# Autodesk Inventor assembly: Bearing Block Assem
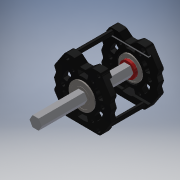
[picture p0: Inventor's stored thumbnail of the model, 180x180]
Saved by Autodesk Inventor 2018 (Build 220112000, 112)
## iProperties
Created: 2018-11-11
Part Number: Bearing Block Assem
Document SubType Name: Assembly
Designer: maste
Author: maste
## Documents named in this file (8)
- F:\Summer Drive Base V1\Summer Drivebase\Bearing Block Assem.iam
- F:\Summer Drive Base V1\Summer Drivebase\VersaBlock_Kit_217-3432.ipt
- F:\Summer Drive Base V1\Summer Drivebase\Ignore this-For constraining purposes.ipt
- F:\Summer Drive Base V1\Summer Drivebase\Pretend this is a bolt.ipt
- F:\Summer Drive Base V1\Summer Drivebase\0_500_Hex_ID_x_1_125_OD_x_0_313_WD_Flanged_Bearing_v2_217-3875.ipt
- F:\Summer Drive Base V1\Summer Drivebase\am-1238+Collar+Clamp,+0.5''+Hex+Bore,+Aluminum.iam
- F:\Summer Drive Base V1\Summer Drivebase\5-1875 hex shaft.ipt
- F:\Summer Drive Base V1\Summer Drivebase\0.125in Spacer.ipt
## Components (12 placed, 7 different names)
1. VersaBlock_Kit_217-3432:1 — Mate:4, Mate:5, Mate:6, Mate:7, Mate:8, Mate:11, Mate:13, Mate:15, Mate:16, Rotation:2
2. VersaBlock_Kit_217-3432:2 — Mate:1, Mate:2, Mate:3, Mate:9, Mate:10, Mate:12, Mate:14, Mate:19, Mate:20, Rotation:1
3. Ignore this-For constraining purposes:3 — Mate:1, Mate:2, Mate:3
4. Pretend this is a bolt:1 — Mate:7, Mate:8, Mate:9, Mate:10
5. Pretend this is a bolt:2 — Mate:11, Mate:12, Mate:13, Mate:14
6. Ignore this-For constraining purposes:4 — Mate:4, Mate:5, Mate:6
7. 0_500_Hex_ID_x_1_125_OD_x_0_313_WD_Flanged_Bearing_v2_217-3875:1 — Mate:15, Mate:16, Mate:17, Flush:1, Flush:2, Rotation:2
8. 0_500_Hex_ID_x_1_125_OD_x_0_313_WD_Flanged_Bearing_v2_217-3875:2 — Mate:18, Flush:3, Flush:4, Mate:19, Mate:20, Rotation:1, Mate:21, Flush:5, Flush:6
9. am-1238+Collar+Clamp,+0.5''+Hex+Bore,+Aluminum:1 [sub-assembly] — Mate:21, Flush:5, Flush:6, Flush:7, Mate:22, Mate:23
10. 5-1875 hex shaft:1 — Flush:7, Mate:22, Mate:23
11. 0.125in Spacer:1 — Mate:17, Flush:1, Flush:2
12. 0.125in Spacer:2 — Mate:18, Flush:3, Flush:4
## Relationships (32: Mate 23, Flush 7, RelateRotation 2)
- Mate:1: VersaBlock_Kit_217-3432:2 ↔ Ignore this-For constraining purposes:3
- Mate:2: VersaBlock_Kit_217-3432:2 ↔ Ignore this-For constraining purposes:3
- Mate:3: VersaBlock_Kit_217-3432:2 ↔ Ignore this-For constraining purposes:3
- Mate:4: VersaBlock_Kit_217-3432:1 ↔ Ignore this-For constraining purposes:4
- Mate:5: VersaBlock_Kit_217-3432:1 ↔ Ignore this-For constraining purposes:4
- Mate:6: VersaBlock_Kit_217-3432:1 ↔ Ignore this-For constraining purposes:4
- Mate:7: VersaBlock_Kit_217-3432:1 ↔ Pretend this is a bolt:1
- Mate:8: VersaBlock_Kit_217-3432:1 ↔ Pretend this is a bolt:1
- Mate:9: VersaBlock_Kit_217-3432:2 ↔ Pretend this is a bolt:1
- Mate:10: VersaBlock_Kit_217-3432:2 ↔ Pretend this is a bolt:1
- Mate:11: VersaBlock_Kit_217-3432:1 ↔ Pretend this is a bolt:2
- Mate:12: VersaBlock_Kit_217-3432:2 ↔ Pretend this is a bolt:2
- Mate:13: VersaBlock_Kit_217-3432:1 ↔ Pretend this is a bolt:2
- Mate:14: VersaBlock_Kit_217-3432:2 ↔ Pretend this is a bolt:2
- Mate:15: VersaBlock_Kit_217-3432:1 ↔ 0_500_Hex_ID_x_1_125_OD_x_0_313_WD_Flanged_Bearing_v2_217-3875:1
- Mate:16: VersaBlock_Kit_217-3432:1 ↔ 0_500_Hex_ID_x_1_125_OD_x_0_313_WD_Flanged_Bearing_v2_217-3875:1
- Mate:17: 0_500_Hex_ID_x_1_125_OD_x_0_313_WD_Flanged_Bearing_v2_217-3875:1 ↔ 0.125in Spacer:1
- Flush:1: 0_500_Hex_ID_x_1_125_OD_x_0_313_WD_Flanged_Bearing_v2_217-3875:1 ↔ 0.125in Spacer:1
- Flush:2: 0_500_Hex_ID_x_1_125_OD_x_0_313_WD_Flanged_Bearing_v2_217-3875:1 ↔ 0.125in Spacer:1
- Mate:18: 0_500_Hex_ID_x_1_125_OD_x_0_313_WD_Flanged_Bearing_v2_217-3875:2 ↔ 0.125in Spacer:2
- Flush:3: 0_500_Hex_ID_x_1_125_OD_x_0_313_WD_Flanged_Bearing_v2_217-3875:2 ↔ 0.125in Spacer:2
- Flush:4: 0_500_Hex_ID_x_1_125_OD_x_0_313_WD_Flanged_Bearing_v2_217-3875:2 ↔ 0.125in Spacer:2
- Mate:19: VersaBlock_Kit_217-3432:2 ↔ 0_500_Hex_ID_x_1_125_OD_x_0_313_WD_Flanged_Bearing_v2_217-3875:2
- Mate:20: VersaBlock_Kit_217-3432:2 ↔ 0_500_Hex_ID_x_1_125_OD_x_0_313_WD_Flanged_Bearing_v2_217-3875:2
- Rotation:1 [RelateRotation] (1 ul): VersaBlock_Kit_217-3432:2 ↔ 0_500_Hex_ID_x_1_125_OD_x_0_313_WD_Flanged_Bearing_v2_217-3875:2
- Rotation:2 [RelateRotation] (1 ul): VersaBlock_Kit_217-3432:1 ↔ 0_500_Hex_ID_x_1_125_OD_x_0_313_WD_Flanged_Bearing_v2_217-3875:1
- Mate:21: 0_500_Hex_ID_x_1_125_OD_x_0_313_WD_Flanged_Bearing_v2_217-3875:2 ↔ am-1238+Collar+Clamp,+0.5''+Hex+Bore,+Aluminum:1
- Flush:5: 0_500_Hex_ID_x_1_125_OD_x_0_313_WD_Flanged_Bearing_v2_217-3875:2 ↔ am-1238+Collar+Clamp,+0.5''+Hex+Bore,+Aluminum:1
- Flush:6: 0_500_Hex_ID_x_1_125_OD_x_0_313_WD_Flanged_Bearing_v2_217-3875:2 ↔ am-1238+Collar+Clamp,+0.5''+Hex+Bore,+Aluminum:1
- Flush:7: am-1238+Collar+Clamp,+0.5''+Hex+Bore,+Aluminum:1 ↔ 5-1875 hex shaft:1
- Mate:22: am-1238+Collar+Clamp,+0.5''+Hex+Bore,+Aluminum:1 ↔ 5-1875 hex shaft:1
- Mate:23: am-1238+Collar+Clamp,+0.5''+Hex+Bore,+Aluminum:1 ↔ 5-1875 hex shaft:1
